# Autodesk Inventor assembly: osszeallitas
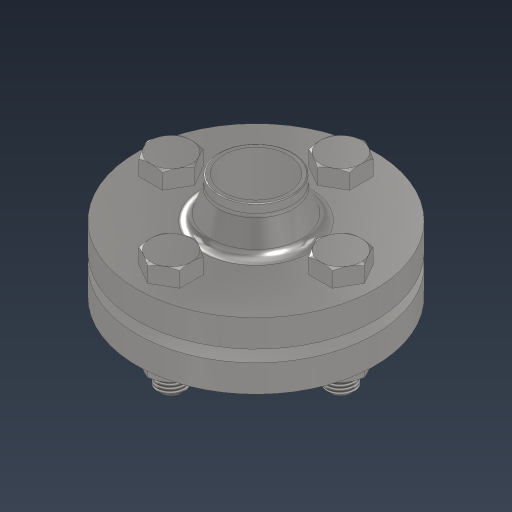
[picture p0: Inventor's stored thumbnail of the model, 512x512]
Saved by Autodesk Inventor 2024.3 (Build 283343000, 343)
## iProperties
Created: 2025-10-06
Part Number: osszeallitas
Document SubType Name: Assembly
Designer: Agi
Author: Agi
## Documents named in this file (6)
- C:\Users\Agi\Desktop\Egyetem\Harmadik félév\Gépelemek\Gépelemek_HF1\Inventor\osszeallitas.iam
- C:\Users\Agi\Desktop\Egyetem\Harmadik félév\Gépelemek\Gépelemek_HF1\Inventor\csavar.ipt
- C:\Users\Agi\Desktop\Egyetem\Harmadik félév\Gépelemek\Gépelemek_HF1\Inventor\csavaranya.ipt
- C:\Users\Agi\Desktop\Egyetem\Harmadik félév\Gépelemek\Gépelemek_HF1\Inventor\karima.ipt
- C:\Users\Agi\Desktop\Egyetem\Harmadik félév\Gépelemek\Gépelemek_HF1\Inventor\tomites.ipt
- C:\Users\Agi\Desktop\Egyetem\Harmadik félév\Gépelemek\Gépelemek_HF1\Inventor\vakkarima.ipt
## Components (11 placed, 5 different names)
1. karima:1 — Mate:1, Mate:2, Mate:3, Mate:4, Mate:6, Mate:7, Mate:8, Mate:9, Mate:12
2. tomites:1 — Mate:1, Mate:2, Mate:3, Mate:5
3. vakkarima:1 — Mate:4, Mate:5, Mate:6, Mate:11
4. csavar:1 — Mate:7, Mate:8, Mate:9, Mate:10
5. csavar:2
6. csavar:3
7. csavar:4
8. csavaranya:1 — Mate:10, Mate:11, Mate:12
9. csavaranya:2
10. csavaranya:3
11. csavaranya:4
## Component patterns: (4 elements, first: csavar:1), (4 elements, first: csavaranya:1)
## Relationships (12: Mate 12)
- Mate:1: karima:1 ↔ tomites:1
- Mate:2: karima:1 ↔ tomites:1
- Mate:3: karima:1 ↔ tomites:1
- Mate:4: karima:1 ↔ vakkarima:1
- Mate:5: tomites:1 ↔ vakkarima:1
- Mate:6: karima:1 ↔ vakkarima:1
- Mate:7: karima:1 ↔ csavar:1
- Mate:8: karima:1 ↔ csavar:1
- Mate:9: karima:1 ↔ csavar:1
- Mate:10: csavar:1 ↔ csavaranya:1
- Mate:11: vakkarima:1 ↔ csavaranya:1
- Mate:12: karima:1 ↔ csavaranya:1
